# Autodesk Inventor assembly: ILO-Mounted
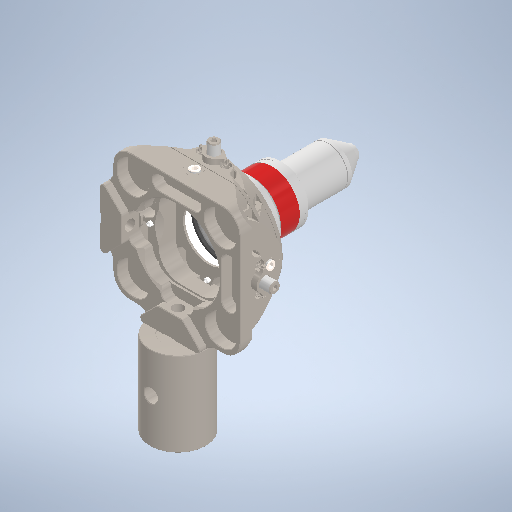
[picture p0: Inventor's stored thumbnail of the model, 512x512]
Saved by Autodesk Inventor 2025.2 (Build 292293000, 293)
## iProperties
Created: 2024-11-27
Part Number: ILO-Mounted
Document SubType Name: Assembly
Designer: monolithic
Author: monolithic
## Documents named in this file (5)
- C:\Users\monolithic\Documents\GitHub\CAD\Monolith\John\Altair_PowellBaseplate_SPIM_ASLM_CTASLM\Assembly\SubAssemblies\ILO-Mounted.iam
- C:\Users\monolithic\Documents\GitHub\CAD\Monolith\John\Altair_PowellBaseplate_SPIM_ASLM_CTASLM\Assembly\SubAssemblies\PLS-P150.ipt
- C:\Users\monolithic\Documents\GitHub\CAD\Monolith\John\Altair_PowellBaseplate_SPIM_ASLM_CTASLM\Assembly\SubAssemblies\POLARIS-1XY.ipt
- C:\Users\monolithic\Documents\GitHub\CAD\Monolith\John\Altair_PowellBaseplate_SPIM_ASLM_CTASLM\Assembly\SubAssemblies\TL20X-MPL.ipt
- C:\Users\monolithic\Documents\GitHub\CAD\Monolith\John\Altair_PowellBaseplate_SPIM_ASLM_CTASLM\Assembly\SubAssemblies\SM1A12.ipt
## Components (4 placed, 4 different names)
1. PLS-P150:1 — Mate:1, Mate:2
2. POLARIS-1XY:1 — Mate:1, Mate:2, Mate:3, Mate:4
3. SM1A12:1 — Mate:3, Mate:4, Mate:5, Mate:6
4. TL20X-MPL:1 — Mate:5, Mate:6
## Relationships (6: Mate 6)
- Mate:1: PLS-P150:1 ↔ POLARIS-1XY:1
- Mate:2: PLS-P150:1 ↔ POLARIS-1XY:1
- Mate:3: POLARIS-1XY:1 ↔ SM1A12:1
- Mate:4: POLARIS-1XY:1 ↔ SM1A12:1
- Mate:5: SM1A12:1 ↔ TL20X-MPL:1
- Mate:6: SM1A12:1 ↔ TL20X-MPL:1
